# Autodesk Inventor assembly: FE Violet Mk V
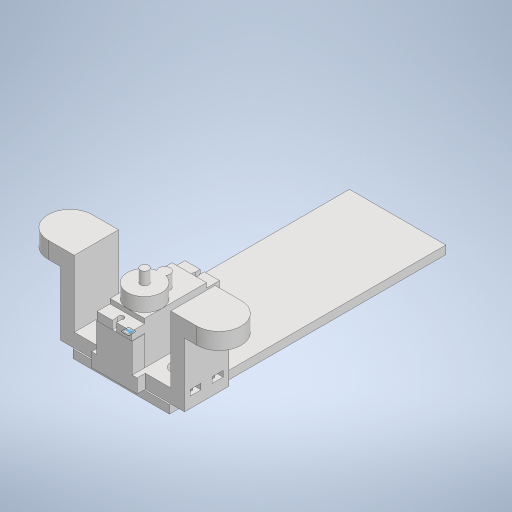
[picture p0: Inventor's stored thumbnail of the model, 512x512]
Saved by Autodesk Inventor 2023 (Build 270158000, 158)
## iProperties
Created: 2023-05-15
Part Number: FE Violet Mk V
Document SubType Name: Assembly
Designer: ivanc
Author: ivanc
## Documents named in this file (4)
- D:\Projects\Robots\FutureEngineers2023_Violet\Models\FE Violet Mk V.iam
- D:\Projects\Robots\FutureEngineers2023_Violet\Models\Enclosure components\Basis of the robot.ipt
- D:\Projects\Robots\FutureEngineers2023_Violet\Models\Electrical components\Servo SG90s.ipt
- D:\Projects\Robots\FutureEngineers2023_Violet\Models\Enclosure components\Basis of steering.ipt
## Components (3 placed, 3 different names)
1. Basis of the robot:1 — Жесткий:1
2. Servo SG90s:1 — Жесткий:2
3. Basis of steering:1 — Жесткий:1, Жесткий:2
## Relationships (2: WeldJoint 2)
- Жесткий:1 [WeldJoint]: Basis of the robot:1 ↔ Basis of steering:1
- Жесткий:2 [WeldJoint]: Servo SG90s:1 ↔ Basis of steering:1
